# Autodesk Inventor assembly: motorAssembly
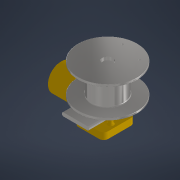
[picture p0: Inventor's stored thumbnail of the model, 180x180]
Saved by Autodesk Inventor 2021 (Build 250183000, 183)
## iProperties
Created: 2021-06-20
Part Number: motorAssembly
Document SubType Name: Assembly
Designer: Watchdog
Mass: 4619.73 g
Surface Area: 1243.51 cm^2
Volume: 874.966 cm^3
Density: 5.27989 g/cm^3
Author: Watchdog
## Documents named in this file (4)
- C:\Users\Watchdog\OneDrive - Flinders\Advn Mech Design Shared\6_Development\2_Design\inventor\support\reel\motorAssembly.iam
- C:\Users\Watchdog\OneDrive - Flinders\Advn Mech Design Shared\6_Development\2_Design\inventor\support\reel\motor.ipt
- C:\Users\Watchdog\OneDrive - Flinders\Advn Mech Design Shared\6_Development\2_Design\inventor\support\reel\reel.ipt
- C:\Users\Watchdog\OneDrive - Flinders\Advn Mech Design Shared\6_Development\2_Design\inventor\support\reel\motorHolder_rotor.ipt
## Components (3 placed, 3 different names)
1. motor:1 — Mate:7, Mate:8, Mate:9, Mate:12, Mate:13, Mate:14
2. reel:1 — Mate:7, Mate:8, Mate:9
3. motorHolder_rotor:1 — Mate:12, Mate:13, Mate:14
## Relationships (6: Mate 6)
- Mate:7: motor:1 ↔ reel:1
- Mate:8: motor:1 ↔ reel:1
- Mate:9: motor:1 ↔ reel:1
- Mate:12: motor:1 ↔ motorHolder_rotor:1
- Mate:13: motor:1 ↔ motorHolder_rotor:1
- Mate:14: motor:1 ↔ motorHolder_rotor:1
